# Autodesk Inventor assembly: FS_kite
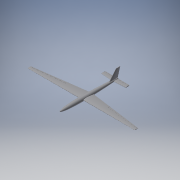
[picture p0: Inventor's stored thumbnail of the model, 180x180]
Saved by Autodesk Inventor 2019 (Build 230136000, 136)
## iProperties
Created: 2019-06-24
Part Number: FS_kite
Document SubType Name: Assembly
Designer: asiddiq2
Mass: 2.33852e+06 g
Surface Area: 431480 cm^2
Volume: 2.33852e+06 cm^3
Density: 1 g/cm^3
Project: DoE MHK
Description: Full-scale kite model
Author: asiddiq2
Title: Full scale kite
## Documents named in this file (5)
- D:\Work\DoEOceanKiteProject\compositions\plants\components\vehicle\vehicleLE\library\ayazAirborneVhcl\CAD\FS_kite.iam
- D:\Work\DoEOceanKiteProject\compositions\plants\components\vehicle\vehicleLE\library\ayazAirborneVhcl\CAD\FS_wing.ipt
- D:\Work\DoEOceanKiteProject\compositions\plants\components\vehicle\vehicleLE\library\ayazAirborneVhcl\CAD\FS_hStab.ipt
- D:\Work\DoEOceanKiteProject\compositions\plants\components\vehicle\vehicleLE\library\ayazAirborneVhcl\CAD\FS_vStab.ipt
- D:\Work\DoEOceanKiteProject\compositions\plants\components\vehicle\vehicleLE\library\ayazAirborneVhcl\CAD\FS_fuselage.ipt
## Components (4 placed, 4 different names)
1. FS_wing:1 — Flush:1, Flush:2, Flush:3, Flush:9
2. FS_hStab:1 — Flush:4, Flush:5, Flush:7, Flush:8, Flush:9
3. FS_vStab:1 — Flush:6, Flush:7, Mate:1
4. FS_fuselage:1 — Mate:2, Mate:3, Mate:4, Flush:8
## Relationships (13: Flush 9, Mate 4)
- Flush:1: FS_wing:1
- Flush:2: FS_wing:1
- Flush:3: FS_wing:1
- Flush:4: FS_hStab:1
- Flush:5: FS_hStab:1
- Flush:6: FS_vStab:1
- Flush:7: FS_hStab:1 ↔ FS_vStab:1
- Mate:1: FS_vStab:1
- Mate:2: FS_fuselage:1
- Mate:3: FS_fuselage:1
- Mate:4: FS_fuselage:1
- Flush:8: FS_hStab:1 ↔ FS_fuselage:1
- Flush:9 (-4071 mm): FS_wing:1 ↔ FS_hStab:1
## Named parameters: k_scale = 1, nom_chord = 1000 mm, perc_HS_le = 4.071, HS_le = 4071 mm
